# Autodesk Inventor assembly: AntiBacklash
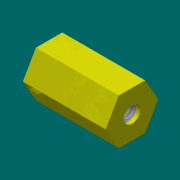
[picture p0: Inventor's stored thumbnail of the model, 180x180]
Saved by Autodesk Inventor 2016 (Build 200138000, 138)
## iProperties
Created: 2015-06-03
Part Number: AntiBacklash
Document SubType Name: Assembly
Designer: Sawaiz Syed
Author: Sawaiz Syed
## Documents named in this file (3)
- C:\Users\Sawaiz\Documents\data\projects\cncBlackBox\xAxis\antiBacklashNut.iam
- C:\Users\Sawaiz\Documents\data\projects\cncBlackBox\hardware\hexNut5-16.ipt
- C:\Users\Sawaiz\Documents\data\projects\cncBlackBox\xAxis\antiBacklashNut.ipt
## Components (3 placed, 2 different names)
1. antiBacklashNut:1 — Mate:2, Mate:3, Flush:1
2. hexNut5-16:1 — Mate:1, Flush:1
3. hexNut5-16:2 — Mate:1, Mate:2, Mate:3
## Relationships (4: Mate 3, Flush 1)
- Mate:1: hexNut5-16:1 ↔ hexNut5-16:2
- Mate:2: antiBacklashNut:1 ↔ hexNut5-16:2
- Mate:3: antiBacklashNut:1 ↔ hexNut5-16:2
- Flush:1: antiBacklashNut:1 ↔ hexNut5-16:1
